# Autodesk Inventor assembly: Assembly2
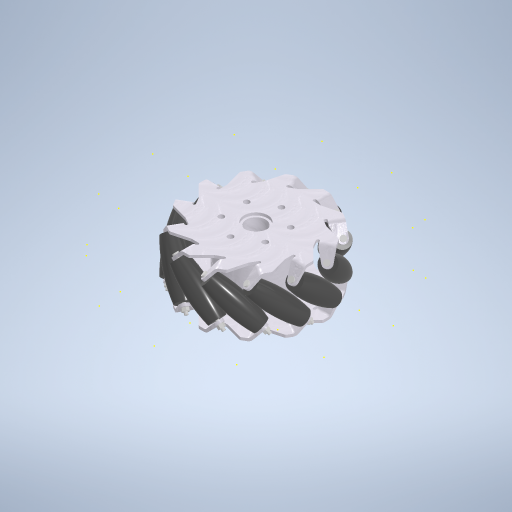
[picture p0: Inventor's stored thumbnail of the model, 512x512]
Saved by Autodesk Inventor 2024 (Build 280153000, 153)
## iProperties
Created: 2023-12-18
Part Number: Assembly2
Document SubType Name: Assembly
Designer: SAHITYA
Author: SAHITYA
## Documents named in this file (5)
- C:\Users\SAHITYA\Documents\Robotics Club (Recruitment_Mechanical)\Mechanum Wheel\Mechanum Wheel.iam
- C:\Users\SAHITYA\Documents\Robotics Club (Recruitment_Mechanical)\Mechanum Wheel\Part1.ipt
- C:\Users\SAHITYA\Documents\Robotics Club (Recruitment_Mechanical)\Mechanum Wheel\Part5.ipt
- C:\Users\SAHITYA\Documents\Robotics Club (Recruitment_Mechanical)\Mechanum Wheel\Part7.ipt
- C:\Users\SAHITYA\Documents\Robotics Club (Recruitment_Mechanical)\Mechanum Wheel\Part8.ipt
## Components (38 placed, 4 different names)
1. Part1:1 — Mate:2, Mate:3, Mate:5, Mate:9, Mate:12
2. Part1:2 — Mate:2, Mate:3, Mate:5, Mate:6, Mate:10
3. Part8:1 — Mate:10
4. Part8:2
5. Part8:3
6. Part8:4
7. Part8:5
8. Part8:6
9. Part8:7
10. Part8:8
11. Part8:9
12. Part8:10
13. Part8:11
14. Part8:12
15. Part5:1 — Mate:6, Mate:9, Mate:11
16. Part7:1 — Mate:11, Mate:12
17. Part5:2
18. Part7:2
19. Part5:3
20. Part7:3
21. Part5:4
22. Part7:4
23. Part5:5
24. Part7:5
25. Part5:6
26. Part7:6
27. Part5:7
28. Part7:7
29. Part5:8
30. Part7:8
31. Part5:9
32. Part7:9
33. Part5:10
34. Part7:10
35. Part5:11
36. Part7:11
37. Part5:12
38. Part7:12
## Component patterns: (12 elements, first: Part8:1), (12 elements, first: Part5:1 + Part7:1)
## Relationships (8: Mate 8)
- Mate:2: Part1:1 ↔ Part1:2
- Mate:3: Part1:1 ↔ Part1:2
- Mate:5: Part1:1 ↔ Part1:2
- Mate:6: Part1:2 ↔ Part5:1
- Mate:9 (0.5 mm): Part1:1 ↔ Part5:1
- Mate:10: Part1:2 ↔ Part8:1
- Mate:11: Part5:1 ↔ Part7:1
- Mate:12: Part1:1 ↔ Part7:1
